# Autodesk Inventor assembly: Asta_verticale
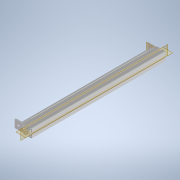
[picture p0: Inventor's stored thumbnail of the model, 180x180]
Saved by Autodesk Inventor 2022 (Build 260153000, 153)
## iProperties
RuleStatus: InUse
Created: 2022-02-11
Part Number: Asta_verticale
Document SubType Name: Assembly
Designer: matte
Author: matte
## Documents named in this file (4)
- C:\Users\matte\Documents\GitHub\MDM-CyberOrto-CAD\Assiemi\Asta_verticale.iam
- C:\Users\matte\Documents\GitHub\MDM-CyberOrto-CAD\Pezzi singoli\Torretta\10-540.ipt
- C:\Users\matte\Documents\GitHub\MDM-CyberOrto-CAD\Parker components\03-Brackets_Gussets_Plates\08-Angle Brackets\28-602.ipt
- C:\Users\matte\Documents\GitHub\MDM-CyberOrto-CAD\Pezzi singoli\Torretta\PowerScrew.ipt
## Components (4 placed, 3 different names)
1. 10-540:1 — Coincidente:1, Allineato:1, Coincidente:2, Coincidente:4, Allineato:4, Coincidente:5
2. 28-602:1 — Coincidente:1, Allineato:1, Coincidente:2, Coincidente:3, Angolo:1
3. PowerScrew:1 — Allineato:2, Allineato:3
4. 28-602:2 — Coincidente:4, Allineato:4, Coincidente:5
## Relationships (10: Mate 5, Flush 4, Angle 1)
- Coincidente:1 [Mate]: 10-540:1 ↔ 28-602:1
- Allineato:1 [Flush]: 10-540:1 ↔ 28-602:1
- Coincidente:2 [Mate]: 10-540:1 ↔ 28-602:1
- Coincidente:3 [Mate]: 28-602:1
- Angolo:1 [Angle] (0 deg): 28-602:1
- Allineato:2 [Flush]: PowerScrew:1
- Allineato:3 [Flush]: PowerScrew:1
- Coincidente:4 [Mate]: 10-540:1 ↔ 28-602:2
- Allineato:4 [Flush]: 10-540:1 ↔ 28-602:2
- Coincidente:5 [Mate]: 10-540:1 ↔ 28-602:2
